# Autodesk Inventor assembly: Scananlage
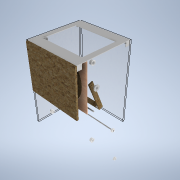
[picture p0: Inventor's stored thumbnail of the model, 180x180]
Saved by Autodesk Inventor 2021 (Build 250183000, 183)
## iProperties
Created: 2022-06-25
Part Number: Scananlage
Document SubType Name: Assembly
Designer: adria
Mass: 14409.4 g
Surface Area: 38340.3 cm^2
Volume: 23914.3 cm^3
Density: 0.602544 g/cm^3
Author: adria
## Documents named in this file (22)
- C:\Users\adria\OneDrive - tum.de\G2_Waste-Recycling\CAD\Scananlage.iam
- C:\Users\adria\OneDrive - tum.de\G2_Waste-Recycling\CAD\Drehteller.ipt
- C:\Users\adria\OneDrive - tum.de\G2_Waste-Recycling\CAD\stepper-motor-nema17-simplified-model-1.snapshot.3\motor.ipt
- C:\Users\adria\OneDrive - tum.de\G2_Waste-Recycling\CAD\Boden.ipt
- C:\Users\adria\OneDrive - tum.de\G2_Waste-Recycling\CAD\Ecken_Box.ipt
- C:\Users\adria\OneDrive - tum.de\G2_Waste-Recycling\CAD\Adapter_Drehteller.ipt
- C:\Users\adria\OneDrive - tum.de\G2_Waste-Recycling\CAD\Clutch_nema.ipt
- C:\Users\adria\OneDrive - tum.de\G2_Waste-Recycling\CAD\Seite.ipt
- C:\Users\adria\OneDrive - tum.de\G2_Waste-Recycling\CAD\Motorstange.ipt
- C:\Users\adria\OneDrive - tum.de\G2_Waste-Recycling\CAD\Rolle_schieber.ipt
- C:\Users\adria\OneDrive - tum.de\G2_Waste-Recycling\CAD\Stange.ipt
- C:\Users\adria\OneDrive - tum.de\G2_Waste-Recycling\CAD\Seite_links.ipt
- C:\Users\adria\OneDrive - tum.de\G2_Waste-Recycling\CAD\Oben.ipt
- C:\Users\adria\OneDrive - tum.de\G2_Waste-Recycling\CAD\Stange_SCHIEBER.ipt
- C:\Users\adria\OneDrive - tum.de\G2_Waste-Recycling\CAD\Hebel_camera.ipt
- C:\Users\adria\OneDrive - tum.de\G2_Waste-Recycling\CAD\Querstrebe_camera.ipt
- C:\Users\adria\OneDrive - tum.de\G2_Waste-Recycling\CAD\Camera.ipt
- C:\Users\adria\OneDrive - tum.de\G2_Waste-Recycling\CAD\Hinterwand.ipt
- C:\Users\adria\OneDrive - tum.de\G2_Waste-Recycling\CAD\Boden_drehscheibe.ipt
- C:\Users\adria\OneDrive - tum.de\G2_Waste-Recycling\CAD\Beschlag_camera.ipt
- C:\Users\adria\OneDrive - tum.de\G2_Waste-Recycling\CAD\GT2 Timing Pulley T40.ipt
- C:\Users\adria\OneDrive - tum.de\G2_Waste-Recycling\CAD\Cameralager22.2mitloecher.ipt
## Components (32 placed, 21 different names)
1. Drehteller:1 — Passend:9, Passend:10, Passend:11, Fluchtend:15
2. motor:1 — Passend:5, Passend:6, Passend:58, Passend:59, Passend:60
3. Boden:1 — Passend:1, Passend:14, Passend:58, Passend:59, Passend:60, Passend:73, Passend:74, Passend:75, Fluchtend:16
4. Adapter_Drehteller:1 — Passend:7, Passend:8, Passend:9, Passend:10, Passend:11
5. Clutch_nema:1 — Passend:5, Passend:6, Passend:7, Passend:8
6. Ecken_Box:1 — Passend:14, Passend:38, Passend:69, Fluchtend:11, Passend:75
7. Seite:1 — Passend:22, Passend:23, Passend:28, Passend:29, Passend:30, Passend:32, Passend:43, Passend:44, Passend:45, Passend:46, Passend:70, Passend:71, Passend:72, Fluchtend:12, Passend:76, Passend:77, Fluchtend:14
8. Motorstange:1 — Passend:32, Passend:43
9. Rolle_schieber:1 — Passend:22, Passend:44
10. Rolle_schieber:2 — Passend:23, Passend:45
11. Rolle_schieber:3 — Passend:81, Passend:82
12. Rolle_schieber:4 — Passend:79, Passend:80
13. motor:2 — Passend:28, Passend:29, Passend:30
14. Motorstange:2 — Passend:41, Passend:83
15. Stange:1 — Passend:83, Fluchtend:14
16. Ecken_Box:8 — Passend:46, Passend:52, Fluchtend:3, Passend:53, Passend:70, Passend:84
17. Seite_links:1 — Passend:38, Passend:41, Passend:54, Passend:69, Fluchtend:11, Fluchtend:13, Passend:79, Passend:80, Passend:81, Passend:82, Passend:87, Passend:92, Passend:93, Passend:94
18. Oben:1 — Passend:52, Fluchtend:3, Passend:53, Passend:55, Passend:56
19. Stange_SCHIEBER:1
20. Ecken_Box:9 — Passend:54, Passend:55, Passend:56, Fluchtend:13
21. Hebel_camera:1 — Passend:64, Fluchtend:5, Fluchtend:6, Passend:89, Fluchtend:17
22. Hebel_camera:2 — Passend:65, Fluchtend:7, Fluchtend:8, Fluchtend:10, Passend:78, Passend:90
23. Querstrebe_camera:1 — Passend:64, Fluchtend:5, Fluchtend:6, Passend:65, Fluchtend:7, Fluchtend:8, Passend:67, Fluchtend:9, Passend:88, Fluchtend:18, Passend:91
24. Camera:1 — Passend:67, Fluchtend:9, Fluchtend:10
25. Ecken_Box:10 — Passend:71, Passend:72, Passend:73, Passend:74, Fluchtend:12, Passend:85, Passend:86
26. motor:4 — Passend:76, Passend:77, Passend:78
27. Hinterwand:1 — Passend:84, Passend:85, Passend:86
28. Boden_drehscheibe:1 — Fluchtend:15, Passend:87, Fluchtend:16
29. Beschlag_camera:1 — Passend:88, Passend:89, Fluchtend:17
30. Beschlag_camera:2 — Fluchtend:18, Passend:90, Passend:91
31. GT2 Timing Pulley T40:1
32. Cameralager22.2mitloecher:1 — Passend:92, Passend:93, Passend:94
## Relationships (73: Mate 58, Flush 15)
- Passend:1 [Mate]: Boden:1
- Passend:5 [Mate]: motor:1 ↔ Clutch_nema:1
- Passend:6 [Mate]: motor:1 ↔ Clutch_nema:1
- Passend:7 [Mate]: Adapter_Drehteller:1 ↔ Clutch_nema:1
- Passend:8 [Mate]: Adapter_Drehteller:1 ↔ Clutch_nema:1
- Passend:9 [Mate]: Drehteller:1 ↔ Adapter_Drehteller:1
- Passend:10 [Mate]: Drehteller:1 ↔ Adapter_Drehteller:1
- Passend:11 [Mate]: Drehteller:1 ↔ Adapter_Drehteller:1
- Passend:14 [Mate]: Boden:1 ↔ Ecken_Box:1
- Passend:22 [Mate]: Seite:1 ↔ Rolle_schieber:1
- Passend:23 [Mate]: Seite:1 ↔ Rolle_schieber:2
- Passend:28 [Mate]: Seite:1 ↔ motor:2
- Passend:29 [Mate]: Seite:1 ↔ motor:2
- Passend:30 [Mate]: Seite:1 ↔ motor:2
- Passend:32 [Mate]: Seite:1 ↔ Motorstange:1
- Passend:38 [Mate]: Ecken_Box:1 ↔ Seite_links:1
- Passend:41 [Mate]: Motorstange:2 ↔ Seite_links:1
- Passend:43 [Mate]: Seite:1 ↔ Motorstange:1
- Passend:44 [Mate]: Seite:1 ↔ Rolle_schieber:1
- Passend:45 [Mate]: Seite:1 ↔ Rolle_schieber:2
- Passend:46 [Mate]: Seite:1 ↔ Ecken_Box:8
- Passend:52 [Mate]: Ecken_Box:8 ↔ Oben:1
- Fluchtend:3 [Flush]: Ecken_Box:8 ↔ Oben:1
- Passend:53 [Mate]: Ecken_Box:8 ↔ Oben:1
- Passend:54 [Mate]: Seite_links:1 ↔ Ecken_Box:9
- Passend:55 [Mate]: Oben:1 ↔ Ecken_Box:9
- Passend:56 [Mate]: Oben:1 ↔ Ecken_Box:9
- Passend:58 [Mate]: motor:1 ↔ Boden:1
- Passend:59 [Mate]: motor:1 ↔ Boden:1
- Passend:60 [Mate]: motor:1 ↔ Boden:1
- Passend:64 [Mate]: Hebel_camera:1 ↔ Querstrebe_camera:1
- Fluchtend:5 [Flush]: Hebel_camera:1 ↔ Querstrebe_camera:1
- Fluchtend:6 [Flush]: Hebel_camera:1 ↔ Querstrebe_camera:1
- Passend:65 [Mate]: Hebel_camera:2 ↔ Querstrebe_camera:1
- Fluchtend:7 [Flush]: Hebel_camera:2 ↔ Querstrebe_camera:1
- Fluchtend:8 [Flush]: Hebel_camera:2 ↔ Querstrebe_camera:1
- Passend:67 [Mate]: Querstrebe_camera:1 ↔ Camera:1
- Fluchtend:9 [Flush]: Querstrebe_camera:1 ↔ Camera:1
- Fluchtend:10 [Flush] (-220 mm): Hebel_camera:2 ↔ Camera:1
- Passend:69 [Mate]: Ecken_Box:1 ↔ Seite_links:1
- Fluchtend:11 [Flush]: Ecken_Box:1 ↔ Seite_links:1
- Passend:70 [Mate]: Seite:1 ↔ Ecken_Box:8
- Passend:71 [Mate]: Seite:1 ↔ Ecken_Box:10
- Passend:72 [Mate]: Seite:1 ↔ Ecken_Box:10
- Passend:73 [Mate]: Boden:1 ↔ Ecken_Box:10
- Passend:74 [Mate]: Boden:1 ↔ Ecken_Box:10
- Passend:75 [Mate]: Boden:1 ↔ Ecken_Box:1
- Fluchtend:12 [Flush]: Seite:1 ↔ Ecken_Box:10
- Fluchtend:13 [Flush]: Seite_links:1 ↔ Ecken_Box:9
- Passend:76 [Mate]: Seite:1 ↔ motor:4
- Passend:77 [Mate]: Seite:1 ↔ motor:4
- Passend:78 [Mate]: Hebel_camera:2 ↔ motor:4
- Passend:79 [Mate]: Rolle_schieber:4 ↔ Seite_links:1
- Passend:80 [Mate]: Rolle_schieber:4 ↔ Seite_links:1
- Passend:81 [Mate]: Rolle_schieber:3 ↔ Seite_links:1
- Passend:82 [Mate]: Rolle_schieber:3 ↔ Seite_links:1
- Passend:83 [Mate]: Motorstange:2 ↔ Stange:1
- Fluchtend:14 [Flush] (-5 mm): Seite:1 ↔ Stange:1
- Passend:84 [Mate]: Ecken_Box:8 ↔ Hinterwand:1
- Passend:85 [Mate]: Ecken_Box:10 ↔ Hinterwand:1
- Passend:86 [Mate]: Ecken_Box:10 ↔ Hinterwand:1
- Fluchtend:15 [Flush]: Drehteller:1 ↔ Boden_drehscheibe:1
- Passend:87 [Mate]: Seite_links:1 ↔ Boden_drehscheibe:1
- Fluchtend:16 [Flush]: Boden:1 ↔ Boden_drehscheibe:1
- Passend:88 [Mate]: Querstrebe_camera:1 ↔ Beschlag_camera:1
- Passend:89 [Mate]: Hebel_camera:1 ↔ Beschlag_camera:1
- Fluchtend:17 [Flush]: Hebel_camera:1 ↔ Beschlag_camera:1
- Fluchtend:18 [Flush]: Querstrebe_camera:1 ↔ Beschlag_camera:2
- Passend:90 [Mate]: Hebel_camera:2 ↔ Beschlag_camera:2
- Passend:91 [Mate]: Querstrebe_camera:1 ↔ Beschlag_camera:2
- Passend:92 [Mate]: Seite_links:1 ↔ Cameralager22.2mitloecher:1
- Passend:93 [Mate]: Seite_links:1 ↔ Cameralager22.2mitloecher:1
- Passend:94 [Mate]: Seite_links:1 ↔ Cameralager22.2mitloecher:1
